# Autodesk Inventor assembly: computer assembly
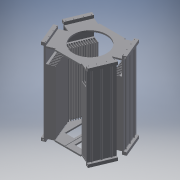
[picture p0: Inventor's stored thumbnail of the model, 180x180]
Saved by Autodesk Inventor 2018 (Build 220112000, 112)
## iProperties
Created: 2018-06-04
Part Number: computer assembly
Document SubType Name: Assembly
Designer: John Viljoen
Author: John Viljoen
## Documents named in this file (7)
- C:\Users\John Viljoen\Documents\Inventor\computer project\computer assembly.iam
- C:\Users\John Viljoen\Documents\Inventor\computer project\baseplate.ipt
- C:\Users\John Viljoen\Documents\Inventor\computer project\coverplate.ipt
- C:\Users\John Viljoen\Documents\Inventor\computer project\topplate.ipt
- C:\Users\John Viljoen\Documents\Inventor\computer project\heat sink.ipt
- C:\Users\John Viljoen\Documents\Inventor\computer project\manifold.ipt
- C:\Users\John Viljoen\Documents\Inventor\computer project\manifold mirror.ipt
## Components (18 placed, 6 different names)
1. baseplate:1 — Mate:9, Flush:5, Flush:6, Mate:11, Mate:13, Mate:15, Mate:17, Mate:20, Flush:12, Mate:24, Flush:14, Mate:30, Flush:17, Mate:32, Flush:18
2. coverplate:1 — Mate:7, Mate:8, Flush:4, Mate:16, Flush:10, Mate:27, Mate:33
3. coverplate:2 — Mate:1, Mate:2, Flush:1, Mate:12, Flush:8, Mate:19, Mate:21
4. coverplate:3 — Mate:5, Mate:6, Flush:3, Mate:9, Flush:5, Flush:6, Mate:14, Flush:9, Mate:23, Mate:25
5. coverplate:4 — Mate:3, Mate:4, Flush:2, Mate:10, Flush:7, Mate:29, Mate:31
6. topplate:1 — Mate:1, Mate:2, Flush:1, Mate:3, Mate:4, Flush:2, Mate:5, Mate:6, Flush:3, Mate:7, Mate:8, Flush:4, Mate:18, Flush:11, Mate:22, Flush:13, Mate:26, Flush:15, Mate:28, Flush:16
7. heat sink:1 — Mate:12, Flush:8, Mate:13
8. heat sink:2 — Mate:14, Flush:9, Mate:15
9. heat sink:3 — Mate:16, Flush:10, Mate:17
10. heat sink:4 — Mate:10, Mate:11, Flush:7
11. manifold:1 — Mate:18, Flush:11, Mate:19
12. manifold:2 — Mate:20, Flush:12, Mate:21
13. manifold:3 — Mate:24, Flush:14, Mate:25
14. manifold:4 — Mate:22, Flush:13, Mate:23
15. manifold mirror:1 — Mate:26, Flush:15, Mate:27
16. manifold mirror:2 — Mate:28, Flush:16, Mate:29
17. manifold mirror:3 — Mate:30, Flush:17, Mate:31
18. manifold mirror:4 — Mate:32, Flush:18, Mate:33
## Relationships (51: Mate 33, Flush 18)
- Mate:1: coverplate:2 ↔ topplate:1
- Mate:2: coverplate:2 ↔ topplate:1
- Flush:1: coverplate:2 ↔ topplate:1
- Mate:3: coverplate:4 ↔ topplate:1
- Mate:4: coverplate:4 ↔ topplate:1
- Flush:2: coverplate:4 ↔ topplate:1
- Mate:5: coverplate:3 ↔ topplate:1
- Mate:6: coverplate:3 ↔ topplate:1
- Flush:3: coverplate:3 ↔ topplate:1
- Mate:7: coverplate:1 ↔ topplate:1
- Mate:8: coverplate:1 ↔ topplate:1
- Flush:4: coverplate:1 ↔ topplate:1
- Mate:9: baseplate:1 ↔ coverplate:3
- Flush:5: baseplate:1 ↔ coverplate:3
- Flush:6: baseplate:1 ↔ coverplate:3
- Mate:10: coverplate:4 ↔ heat sink:4
- Mate:11: baseplate:1 ↔ heat sink:4
- Flush:7: coverplate:4 ↔ heat sink:4
- Mate:12: coverplate:2 ↔ heat sink:1
- Flush:8: coverplate:2 ↔ heat sink:1
- Mate:13: baseplate:1 ↔ heat sink:1
- Mate:14: coverplate:3 ↔ heat sink:2
- Flush:9: coverplate:3 ↔ heat sink:2
- Mate:15: baseplate:1 ↔ heat sink:2
- Mate:16: coverplate:1 ↔ heat sink:3
- Flush:10: coverplate:1 ↔ heat sink:3
- Mate:17: baseplate:1 ↔ heat sink:3
- Mate:18: topplate:1 ↔ manifold:1
- Flush:11: topplate:1 ↔ manifold:1
- Mate:19: coverplate:2 ↔ manifold:1
- Mate:20: baseplate:1 ↔ manifold:2
- Flush:12: baseplate:1 ↔ manifold:2
- Mate:21: coverplate:2 ↔ manifold:2
- Mate:22: topplate:1 ↔ manifold:4
- Flush:13: topplate:1 ↔ manifold:4
- Mate:23: coverplate:3 ↔ manifold:4
- Mate:24: baseplate:1 ↔ manifold:3
- Flush:14: baseplate:1 ↔ manifold:3
- Mate:25: coverplate:3 ↔ manifold:3
- Mate:26: topplate:1 ↔ manifold mirror:1
- Flush:15: topplate:1 ↔ manifold mirror:1
- Mate:27: coverplate:1 ↔ manifold mirror:1
- Mate:28: topplate:1 ↔ manifold mirror:2
- Flush:16: topplate:1 ↔ manifold mirror:2
- Mate:29: coverplate:4 ↔ manifold mirror:2
- Mate:30: baseplate:1 ↔ manifold mirror:3
- Flush:17: baseplate:1 ↔ manifold mirror:3
- Mate:31: coverplate:4 ↔ manifold mirror:3
- Mate:32: baseplate:1 ↔ manifold mirror:4
- Flush:18: baseplate:1 ↔ manifold mirror:4
- Mate:33: coverplate:1 ↔ manifold mirror:4
